# Autodesk Inventor assembly: Ensemble1
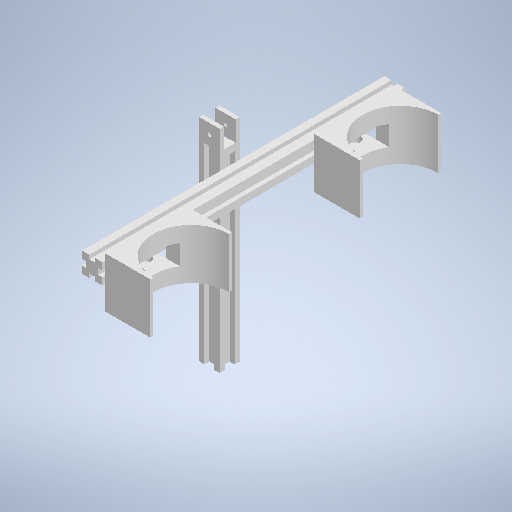
[picture p0: Inventor's stored thumbnail of the model, 512x512]
Saved by Autodesk Inventor 2025 (Build 290162000, 162)
## iProperties
Created: 2024-11-18
Part Number: Ensemble1
Document SubType Name: Assembly
Designer: chass
Author: chass
## Documents named in this file (4)
- C:\Users\chass\Documents\AREM\Robot-CdR-2025\Modeles-3D\actionneur_elevateur\Ensemble1.iam
- C:\Users\chass\Documents\AREM\Robot-CdR-2025\Modeles-3D\actionneur_elevateur\rail_principal.ipt
- C:\Users\chass\Documents\AREM\Robot-CdR-2025\Modeles-3D\actionneur_elevateur\barre_horizontale_support_pinces.ipt
- C:\Users\chass\Documents\AREM\Robot-CdR-2025\Modeles-3D\actionneur_elevateur\corps_pince_aimant.ipt
## Components (4 placed, 3 different names)
1. barre_horizontale_support_pinces:1 — Placage:1, Placage:2, Placage:3, Placage:4
2. corps_pince_aimant:1 — Placage:1, Placage:2
3. corps_pince_aimant:2 — Placage:3
4. rail_principal:1 — Placage:4
## Relationships (4: Mate 4)
- Placage:1 [Mate]: barre_horizontale_support_pinces:1 ↔ corps_pince_aimant:1
- Placage:2 [Mate]: barre_horizontale_support_pinces:1 ↔ corps_pince_aimant:1
- Placage:3 [Mate]: barre_horizontale_support_pinces:1 ↔ corps_pince_aimant:2
- Placage:4 [Mate]: barre_horizontale_support_pinces:1 ↔ rail_principal:1
